# Autodesk Inventor assembly: battery
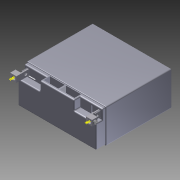
[picture p0: Inventor's stored thumbnail of the model, 180x180]
Saved by Autodesk Inventor 2011 (Build 150239000, 239)
## iProperties
Created: 2010-02-09
Part Number: battery
Document SubType Name: Assembly
Designer: a
Author: a
## Documents named in this file (5)
- R:\2012\Inventor\vkop\All-Electrical\battery.iam
- R:\2012\Inventor\vkop\All-Electrical\Battery_MK_ES17-12.ipt
- R:\2012\Inventor\vkop\All-Electrical\Terminal Lug _Burndy_KPA4C.iam
- C:\Documents and Settings\kysmart\My Documents\Inventor\Content Center Files\R2010\en-US\ANSI B18.2.1(3)\ANSI B18.2.1 - 1_4-20 UNC - 0.5(3).ipt
- C:\Documents and Settings\kysmart\My Documents\Inventor\Content Center Files\R2010\en-US\ANSI B18.2.2(09)\ANSI B18.2.2 - 1_4 - 20(2).ipt
## Components (7 placed, 4 different names)
1. Battery_MK_ES17-12:1 — Mate:1, Angle:1, Mate:2, Mate:3, Mate:4, Angle:2, Mate:6, Mate:8
2. Terminal Lug _Burndy_KPA4C:1 [sub-assembly] — Mate:1, Angle:1, Mate:2, Insert:2
3. Terminal Lug _Burndy_KPA4C:2 [sub-assembly] — Mate:3, Mate:4, Angle:2, Insert:1
4. Hex Cap Screw - Inch 1/4-20 UNC - 0.5:1 — Insert:1, Mate:5
5. Hex Cap Screw - Inch 1/4-20 UNC - 0.5:2 — Insert:2, Mate:7
6. Hex Nut - Inch 1/4 - 20:1 — Mate:5, Mate:6
7. Hex Nut - Inch 1/4 - 20:2 — Mate:7, Mate:8
## Relationships (12: Mate 8, Angle 2, Insert 2)
- Mate:1: Battery_MK_ES17-12:1 ↔ Terminal Lug _Burndy_KPA4C:1
- Angle:1 (0 deg): Battery_MK_ES17-12:1 ↔ Terminal Lug _Burndy_KPA4C:1
- Mate:2: Battery_MK_ES17-12:1 ↔ Terminal Lug _Burndy_KPA4C:1
- Mate:3: Battery_MK_ES17-12:1 ↔ Terminal Lug _Burndy_KPA4C:2
- Mate:4: Battery_MK_ES17-12:1 ↔ Terminal Lug _Burndy_KPA4C:2
- Angle:2 (0 deg): Battery_MK_ES17-12:1 ↔ Terminal Lug _Burndy_KPA4C:2
- Mate:6: Battery_MK_ES17-12:1 ↔ Hex Nut - Inch 1/4 - 20:1
- Mate:8: Battery_MK_ES17-12:1 ↔ Hex Nut - Inch 1/4 - 20:2
- Insert:1 (-12.065 mm): Terminal Lug _Burndy_KPA4C:2 ↔ Hex Cap Screw - Inch 1/4-20 UNC - 0.5:1
- Insert:2 (-12.065 mm): Terminal Lug _Burndy_KPA4C:1 ↔ Hex Cap Screw - Inch 1/4-20 UNC - 0.5:2
- Mate:5: Hex Cap Screw - Inch 1/4-20 UNC - 0.5:1 ↔ Hex Nut - Inch 1/4 - 20:1
- Mate:7: Hex Cap Screw - Inch 1/4-20 UNC - 0.5:2 ↔ Hex Nut - Inch 1/4 - 20:2
